# Autodesk Inventor assembly: FrameV2
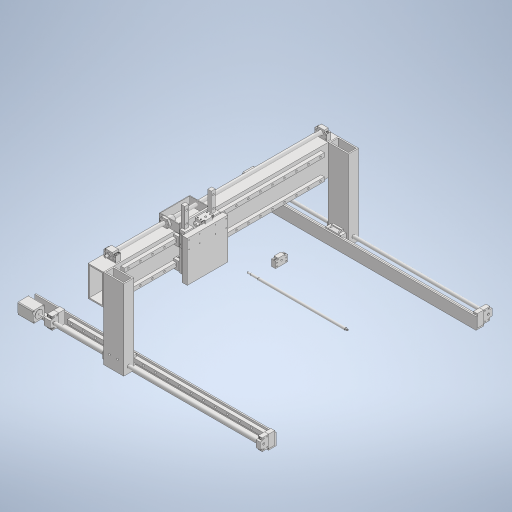
[picture p0: Inventor's stored thumbnail of the model, 512x512]
Saved by Autodesk Inventor 2023 (Build 270158000, 158)
## iProperties
Created: 2022-05-01
Part Number: FrameV2
Document SubType Name: Assembly
Designer: plebbb
Author: plebbb
## Documents named in this file (28)
- D:\Users\plebbb\Desktop\CNC_Project\FrameV2.iam
- D:\Users\plebbb\Desktop\CNC_Project\HGW20CC_Rail_800mm.ipt
- D:\Users\plebbb\Desktop\CNC_Project\HGW20CC_Slider.ipt
- D:\Users\plebbb\Desktop\CNC_Project\SFU1605_800mm.ipt
- D:\Users\plebbb\Desktop\CNC_Project\SFU1605_Nut.ipt
- D:\Users\plebbb\Desktop\CNC_Project\BF12.ipt
- D:\Users\plebbb\Desktop\CNC_Project\BK12.ipt
- D:\Users\plebbb\Desktop\CNC_Project\VERTICALTUBE.ipt
- D:\Users\plebbb\Desktop\CNC_Project\Steel_L_Bracket.ipt
- D:\Users\plebbb\Desktop\CNC_Project\BF12_Spacer.ipt
- D:\Users\plebbb\Desktop\CNC_Project\BK12_Spacer.ipt
- D:\Users\plebbb\Desktop\CNC_Project\Nema23.ipt
- D:\Users\plebbb\Desktop\CNC_Project\VERTICALTUBE_Reverse.ipt
- D:\Users\plebbb\Desktop\CNC_Project\HORIZONTALTUBE.ipt
- D:\Users\plebbb\Desktop\CNC_Project\YGANTRYTUBE.ipt
- D:\Users\plebbb\Desktop\CNC_Project\Y_PLATE.ipt
- D:\Users\plebbb\Desktop\CNC_Project\HGW20CC_Rail_300mm.ipt
- D:\Users\plebbb\Desktop\CNC_Project\Z_PLATE.ipt
- D:\Users\plebbb\Desktop\CNC_Project\SFU1204-500.ipt
- D:\Users\plebbb\Desktop\CNC_Project\SFU1204-Housing.ipt
- D:\Users\plebbb\Desktop\CNC_Project\BF10.ipt
- D:\Users\plebbb\Desktop\CNC_Project\BK10.ipt
- D:\Users\plebbb\Desktop\CNC_Project\FrameV2\AIP\FEA\dykw6qf28.fins
- D:\Users\plebbb\Desktop\CNC_Project\FrameV2\AIP\FEA\dykw6qf28.fsat
- D:\Users\plebbb\Desktop\CNC_Project\FrameV2\AIP\FEA\dykw6qf28.ftes
- D:\Users\plebbb\Desktop\CNC_Project\FrameV2\AIP\FEA\dykw6qf28.fwiz
- D:\Users\plebbb\Desktop\CNC_Project\FrameV2\AIP\FEA\dykw6qfc0.fmsh
- D:\Users\plebbb\Desktop\CNC_Project\FrameV2\AIP\FEA\dykw6qfcw.fres
## Components (44 placed, 21 different names)
1. VERTICALTUBE_Reverse:1 — Mate:64, Mate:65, Mate:66, Mate:72, Mate:76, Mate:79, Mate:83
2. Steel_L_Bracket:2 — Flush:25, Mate:48, Mate:52, Flush:52, Angle:3, Flush:54, Flush:55, Mate:67, Flush:56, Flush:57, Mate:77
3. HGW20CC_Rail_800mm:2 — Flush:25, Mate:48, Mate:59, Mate:60, Mate:75
4. BK12_Spacer:2 — Mate:52, Flush:52, Mate:56, Mate:57, Mate:58
5. BF12:2 — Mate:62, Mate:68, Mate:69, Mate:70, Mate:72
6. BK12:2 — Mate:56, Mate:57, Mate:58, Mate:61, Flush:53
7. SFU1605_800mm:2 — Mate:61, Flush:53, Mate:62, Mate:63, Mate:64, Mate:71, Mate:73, Mate:74
8. HGW20CC_Slider:3 — Mate:59, Mate:60, Mate:76
9. SFU1605_Nut:2 — Mate:63, Angle:3, Mate:65, Mate:66, Mate:71
10. BF12_Spacer:2 — Flush:54, Flush:55, Mate:67, Mate:68, Mate:69, Mate:70, Mate:75
11. Nema23:2 — Mate:73, Mate:74
12. HGW20CC_Rail_800mm:3 — Mate:80, Mate:82, Angle:4, Angle:5, Mate:83, Flush:60, Mate:88, Mate:89, Mate:90, Mate:91, Flush:65, Flush:66
13. HGW20CC_Rail_800mm:4 — Mate:81, Mate:82, Angle:4, Flush:60, Flush:61, Mate:84, Mate:85, Mate:86, Mate:87, Flush:62, Flush:64
14. HORIZONTALTUBE:1 — Mate:78, Mate:79, Flush:58, Flush:59, Mate:80, Mate:81, Angle:5, Flush:61, Mate:94, Flush:68, Flush:69, Mate:95, Angle:6
15. HGW20CC_Slider:4 — Mate:84, Mate:85, Flush:62, Mate:92, Flush:72
16. HGW20CC_Slider:5 — Mate:86, Mate:87, Mate:92, Flush:64, Flush:70, Flush:75
17. HGW20CC_Slider:6 — Mate:88, Mate:90, Mate:93, Flush:66, Flush:74
18. HGW20CC_Slider:7 — Mate:89, Mate:91, Flush:65, Mate:93, Flush:73
19. BF12:3 — Flush:67, Mate:94, Flush:68, Mate:96, Mate:97
20. BK12:3 — Flush:69, Mate:95, Mate:98
21. SFU1605_800mm:3 — Mate:96, Mate:97, Mate:98, Mate:99
22. SFU1605_Nut:3 — Mate:99, Mate:100, Angle:7, Flush:71
23. YGANTRYTUBE:1 — Mate:100, Angle:6, Flush:70, Angle:7, Flush:71, Mate:101, Mate:102, Mate:103, Flush:83
24. Y_PLATE:1 — Mate:101, Mate:102, Mate:103, Flush:72, Flush:73, Flush:74, Flush:75, Mate:104, Mate:105, Angle:9, Flush:76, Flush:78, Flush:79, Angle:10, Mate:113, Mate:115
25. HGW20CC_Rail_300mm:1 — Mate:104, Angle:8, Angle:9, Flush:77, Flush:79, Mate:107, Mate:108
26. HGW20CC_Rail_300mm:3 — Mate:105, Angle:8, Flush:76, Flush:77, Flush:78, Mate:106, Mate:109, Flush:80, Flush:81, Mate:116
27. Z_PLATE:1 — Mate:110, Angle:10, Mate:111, Mate:112, Flush:82, Mate:114
28. HGW20CC_Slider:8 — Mate:106, Mate:109, Mate:110, Mate:111, Flush:80, Flush:81
29. HGW20CC_Slider:9 — Mate:107, Mate:108, Mate:112
30. SFU1204-500:1
31. SFU1204-Housing:1 — Mate:113, Flush:82, Mate:114
32. BF10:1
33. BK10:1 — Mate:115, Mate:116, Flush:83
34. HGW20CC_Rail_800mm:1 — Mate:3, Mate:4, Flush:1, Flush:21, Mate:35, Mate:38
35. SFU1605_800mm:1 — Mate:9, Mate:16, Flush:19, Mate:17, Mate:18, Mate:32, Mate:44, Mate:46, Mate:47
36. SFU1605_Nut:1 — Mate:9, Mate:33, Mate:34, Mate:44
37. HGW20CC_Slider:2 — Mate:3, Mate:4, Flush:1, Mate:25, Mate:30, Mate:31
38. BF12:1 — Mate:17, Mate:18, Angle:1, Mate:37, Mate:45
39. BK12:1 — Mate:16, Flush:19, Angle:2, Mate:40, Mate:41
40. VERTICALTUBE:1 — Mate:25, Mate:30, Mate:31, Mate:32, Mate:33, Mate:34, Mate:45, Mate:78, Flush:58, Flush:59, Flush:67
41. Steel_L_Bracket:1 — Flush:21, Mate:35, Angle:1, Mate:36, Flush:22, Flush:23, Angle:2, Mate:39, Flush:24, Flush:63, Mate:43, Flush:56, Flush:57, Mate:77
42. BF12_Spacer:1 — Mate:36, Flush:22, Flush:23, Mate:37, Mate:38
43. BK12_Spacer:1 — Mate:39, Flush:24, Mate:40, Mate:41
44. Nema23:1 — Mate:46, Mate:47
## Relationships (136: Mate 87, Flush 39, Angle 10)
- Mate:3: HGW20CC_Rail_800mm:1 ↔ HGW20CC_Slider:2
- Mate:4: HGW20CC_Rail_800mm:1 ↔ HGW20CC_Slider:2
- Mate:9: SFU1605_800mm:1 ↔ SFU1605_Nut:1
- Flush:1: HGW20CC_Rail_800mm:1 ↔ HGW20CC_Slider:2
- Mate:16: SFU1605_800mm:1 ↔ BK12:1
- Flush:19: SFU1605_800mm:1 ↔ BK12:1
- Mate:17: SFU1605_800mm:1 ↔ BF12:1
- Mate:18: SFU1605_800mm:1 ↔ BF12:1
- Mate:25: HGW20CC_Slider:2 ↔ VERTICALTUBE:1
- Mate:30: HGW20CC_Slider:2 ↔ VERTICALTUBE:1
- Mate:31: HGW20CC_Slider:2 ↔ VERTICALTUBE:1
- Mate:32: SFU1605_800mm:1 ↔ VERTICALTUBE:1
- Mate:33: SFU1605_Nut:1 ↔ VERTICALTUBE:1
- Mate:34: SFU1605_Nut:1 ↔ VERTICALTUBE:1
- Flush:21 (10 mm): HGW20CC_Rail_800mm:1 ↔ Steel_L_Bracket:1
- Mate:35: HGW20CC_Rail_800mm:1 ↔ Steel_L_Bracket:1
- Angle:1 (0 deg): BF12:1 ↔ Steel_L_Bracket:1
- Mate:36: Steel_L_Bracket:1 ↔ BF12_Spacer:1
- Flush:22: Steel_L_Bracket:1 ↔ BF12_Spacer:1
- Flush:23 (-10 mm): Steel_L_Bracket:1 ↔ BF12_Spacer:1
- Mate:37: BF12:1 ↔ BF12_Spacer:1
- Angle:2 (0 deg): BK12:1 ↔ Steel_L_Bracket:1
- Mate:38: HGW20CC_Rail_800mm:1 ↔ BF12_Spacer:1
- Mate:39: Steel_L_Bracket:1 ↔ BK12_Spacer:1
- Flush:24 (-10 mm): Steel_L_Bracket:1 ↔ BK12_Spacer:1
- Mate:40: BK12:1 ↔ BK12_Spacer:1
- Mate:41: BK12:1 ↔ BK12_Spacer:1
- Flush:63: Steel_L_Bracket:1
- Mate:43: Steel_L_Bracket:1
- Mate:44: SFU1605_800mm:1 ↔ SFU1605_Nut:1
- Mate:45: BF12:1 ↔ VERTICALTUBE:1
- Mate:46: SFU1605_800mm:1 ↔ Nema23:1
- Mate:47: SFU1605_800mm:1 ↔ Nema23:1
- Flush:25 (10 mm): Steel_L_Bracket:2 ↔ HGW20CC_Rail_800mm:2
- Mate:48: Steel_L_Bracket:2 ↔ HGW20CC_Rail_800mm:2
- Mate:52: Steel_L_Bracket:2 ↔ BK12_Spacer:2
- Flush:52 (10 mm): Steel_L_Bracket:2 ↔ BK12_Spacer:2
- Mate:56: BK12_Spacer:2 ↔ BK12:2
- Mate:57: BK12_Spacer:2 ↔ BK12:2
- Mate:58: BK12_Spacer:2 ↔ BK12:2
- Mate:59: HGW20CC_Rail_800mm:2 ↔ HGW20CC_Slider:3
- Mate:60: HGW20CC_Rail_800mm:2 ↔ HGW20CC_Slider:3
- Mate:61: BK12:2 ↔ SFU1605_800mm:2
- Flush:53: BK12:2 ↔ SFU1605_800mm:2
- Mate:62: BF12:2 ↔ SFU1605_800mm:2
- Mate:63: SFU1605_800mm:2 ↔ SFU1605_Nut:2
- Mate:64: VERTICALTUBE_Reverse:1 ↔ SFU1605_800mm:2
- Angle:3 (0 deg): Steel_L_Bracket:2 ↔ SFU1605_Nut:2
- Mate:65: VERTICALTUBE_Reverse:1 ↔ SFU1605_Nut:2
- Mate:66: VERTICALTUBE_Reverse:1 ↔ SFU1605_Nut:2
- Flush:54 (-10 mm): Steel_L_Bracket:2 ↔ BF12_Spacer:2
- Flush:55: Steel_L_Bracket:2 ↔ BF12_Spacer:2
- Mate:67: Steel_L_Bracket:2 ↔ BF12_Spacer:2
- Mate:68: BF12:2 ↔ BF12_Spacer:2
- Mate:69: BF12:2 ↔ BF12_Spacer:2
- Mate:70: BF12:2 ↔ BF12_Spacer:2
- Mate:71: SFU1605_800mm:2 ↔ SFU1605_Nut:2
- Mate:72: VERTICALTUBE_Reverse:1 ↔ BF12:2
- Mate:73: SFU1605_800mm:2 ↔ Nema23:2
- Mate:74: SFU1605_800mm:2 ↔ Nema23:2
- Flush:56: Steel_L_Bracket:2 ↔ Steel_L_Bracket:1
- Mate:75: HGW20CC_Rail_800mm:2 ↔ BF12_Spacer:2
- Flush:57: Steel_L_Bracket:2 ↔ Steel_L_Bracket:1
- Mate:76: VERTICALTUBE_Reverse:1 ↔ HGW20CC_Slider:3
- Mate:77 (1000 mm): Steel_L_Bracket:2 ↔ Steel_L_Bracket:1
- Mate:78: HORIZONTALTUBE:1 ↔ VERTICALTUBE:1
- Mate:79: VERTICALTUBE_Reverse:1 ↔ HORIZONTALTUBE:1
- Flush:58: HORIZONTALTUBE:1 ↔ VERTICALTUBE:1
- Flush:59: HORIZONTALTUBE:1 ↔ VERTICALTUBE:1
- Mate:80: HGW20CC_Rail_800mm:3 ↔ HORIZONTALTUBE:1
- Mate:81: HGW20CC_Rail_800mm:4 ↔ HORIZONTALTUBE:1
- Mate:82 (85 mm): HGW20CC_Rail_800mm:3 ↔ HGW20CC_Rail_800mm:4
- Angle:4 (0 deg): HGW20CC_Rail_800mm:3 ↔ HGW20CC_Rail_800mm:4
- Angle:5 (0 deg): HGW20CC_Rail_800mm:3 ↔ HORIZONTALTUBE:1
- Mate:83 (36.35 mm): VERTICALTUBE_Reverse:1 ↔ HGW20CC_Rail_800mm:3
- Flush:60: HGW20CC_Rail_800mm:3 ↔ HGW20CC_Rail_800mm:4
- Flush:61 (17.5 mm): HGW20CC_Rail_800mm:4 ↔ HORIZONTALTUBE:1
- Mate:84: HGW20CC_Rail_800mm:4 ↔ HGW20CC_Slider:4
- Mate:85: HGW20CC_Rail_800mm:4 ↔ HGW20CC_Slider:4
- Mate:86: HGW20CC_Rail_800mm:4 ↔ HGW20CC_Slider:5
- Mate:87: HGW20CC_Rail_800mm:4 ↔ HGW20CC_Slider:5
- Mate:88: HGW20CC_Rail_800mm:3 ↔ HGW20CC_Slider:6
- Mate:89: HGW20CC_Rail_800mm:3 ↔ HGW20CC_Slider:7
- Mate:90: HGW20CC_Rail_800mm:3 ↔ HGW20CC_Slider:6
- Mate:91: HGW20CC_Rail_800mm:3 ↔ HGW20CC_Slider:7
- Flush:62: HGW20CC_Rail_800mm:4 ↔ HGW20CC_Slider:4
- Mate:92: HGW20CC_Slider:4 ↔ HGW20CC_Slider:5
- Flush:64: HGW20CC_Rail_800mm:4 ↔ HGW20CC_Slider:5
- Flush:65: HGW20CC_Rail_800mm:3 ↔ HGW20CC_Slider:7
- Mate:93: HGW20CC_Slider:6 ↔ HGW20CC_Slider:7
- Flush:66: HGW20CC_Rail_800mm:3 ↔ HGW20CC_Slider:6
- Flush:67: BF12:3 ↔ VERTICALTUBE:1
- Mate:94: HORIZONTALTUBE:1 ↔ BF12:3
- Flush:68 (-10 mm): HORIZONTALTUBE:1 ↔ BF12:3
- Flush:69 (10 mm): HORIZONTALTUBE:1 ↔ BK12:3
- Mate:95: HORIZONTALTUBE:1 ↔ BK12:3
- Mate:96: BF12:3 ↔ SFU1605_800mm:3
- Mate:97: BF12:3 ↔ SFU1605_800mm:3
- Mate:98: BK12:3 ↔ SFU1605_800mm:3
- Mate:99: SFU1605_800mm:3 ↔ SFU1605_Nut:3
- Mate:100: SFU1605_Nut:3 ↔ YGANTRYTUBE:1
- Angle:6 (0 deg): HORIZONTALTUBE:1 ↔ YGANTRYTUBE:1
- Flush:70: HGW20CC_Slider:5 ↔ YGANTRYTUBE:1
- Angle:7 (0 deg): SFU1605_Nut:3 ↔ YGANTRYTUBE:1
- Flush:71: SFU1605_Nut:3 ↔ YGANTRYTUBE:1
- Mate:101: YGANTRYTUBE:1 ↔ Y_PLATE:1
- Mate:102: YGANTRYTUBE:1 ↔ Y_PLATE:1
- Mate:103: YGANTRYTUBE:1 ↔ Y_PLATE:1
- Flush:72 (-5 mm): HGW20CC_Slider:4 ↔ Y_PLATE:1
- Flush:73 (-5 mm): HGW20CC_Slider:7 ↔ Y_PLATE:1
- Flush:74 (-5 mm): HGW20CC_Slider:6 ↔ Y_PLATE:1
- Flush:75 (-5 mm): HGW20CC_Slider:5 ↔ Y_PLATE:1
- Mate:104: Y_PLATE:1 ↔ HGW20CC_Rail_300mm:1
- Mate:105: Y_PLATE:1 ↔ HGW20CC_Rail_300mm:3
- Angle:8 (0 deg): HGW20CC_Rail_300mm:1 ↔ HGW20CC_Rail_300mm:3
- Angle:9 (0 deg): Y_PLATE:1 ↔ HGW20CC_Rail_300mm:1
- Flush:76: Y_PLATE:1 ↔ HGW20CC_Rail_300mm:3
- Flush:77: HGW20CC_Rail_300mm:1 ↔ HGW20CC_Rail_300mm:3
- Flush:78: Y_PLATE:1 ↔ HGW20CC_Rail_300mm:3
- Flush:79: Y_PLATE:1 ↔ HGW20CC_Rail_300mm:1
- Mate:106: HGW20CC_Rail_300mm:3 ↔ HGW20CC_Slider:8
- Mate:107: HGW20CC_Rail_300mm:1 ↔ HGW20CC_Slider:9
- Mate:108: HGW20CC_Rail_300mm:1 ↔ HGW20CC_Slider:9
- Mate:109: HGW20CC_Rail_300mm:3 ↔ HGW20CC_Slider:8
- Mate:110: Z_PLATE:1 ↔ HGW20CC_Slider:8
- Angle:10 (0 deg): Y_PLATE:1 ↔ Z_PLATE:1
- Mate:111: Z_PLATE:1 ↔ HGW20CC_Slider:8
- Mate:112: Z_PLATE:1 ↔ HGW20CC_Slider:9
- Flush:80: HGW20CC_Rail_300mm:3 ↔ HGW20CC_Slider:8
- Flush:81: HGW20CC_Rail_300mm:3 ↔ HGW20CC_Slider:8
- Mate:113: Y_PLATE:1 ↔ SFU1204-Housing:1
- Flush:82: Z_PLATE:1 ↔ SFU1204-Housing:1
- Mate:114 (-101.6 mm): Z_PLATE:1 ↔ SFU1204-Housing:1
- Mate:115: Y_PLATE:1 ↔ BK10:1
- Mate:116 (101.6 mm): HGW20CC_Rail_300mm:3 ↔ BK10:1
- Flush:83: YGANTRYTUBE:1 ↔ BK10:1
## Named parameters: sa_0 = 100000, sa_1 = 50000
note: some values were not read from the file. Shown as the stored number, unit unknown: "sa_0", "sa_1".
